# Autodesk Inventor assembly: 1977000 EAMM-A-D40-60P
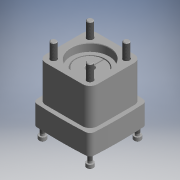
[picture p0: Inventor's stored thumbnail of the model, 180x180]
Saved by Autodesk Inventor 2017.3 (Build 213256000, 256)
## iProperties
Category: PARTsolutions
Company: FESTO
Part Number: 1977000 EAMM-A-D40-60P
Catalog Web Link: www.cadenas.de
Description: EAMM-A-axial kit
Vendor: FESTO
Document SubType Name: Assembly
Designer: partserver
Manufacturer: FESTO
Mass: 430 g
Surface Area: 514.373 cm^2
Volume: 141.907 cm^3
Density: 3.03016 g/cm^3
Title: 1977000 EAMM-A-D40-60P
Author: Cadenas PARTsolutions
Comments: axial kit
PSOL_IDENT_0: {ATYP=ASSISTANT},{DATA=script=$CADENAS_DATA/23d-libs/festo/webfesto.vbb&M_FAMILY=EAMM&M_GROUP=01&M_P
PSOL_IDENT_1: ARTNO=1977000&IDCODE1=EAMM-A-D40-60P&IDCODE2=&customer_number_cns=&MATES=1&LOD=HI&LOCKERP=0&SINGLEPA
PSOL_IDENT_2: RT=1}
NB: 1977000 EAMM-A-D40-60P
NN: EAMM-A
NT: axial kit
NBSYN: $TNR. $TYP.
LINA: 1977000 EAMM-A-D40-60P
CATALOG: Festo
TNR: 1977000
TYP: EAMM-A-D40-60P
CNSMASSEXACT: 0.43
SUPPLIER: FESTO
ARTICLENO: 1977000 EAMM-A-D40-60P
BOMINFO: 1977000 EAMM-A-D40-60P
CREATOR: CADENAS GmbH
## Documents named in this file (7)
- e:\temp\worker_10\temp\exporttempdir_3840_10_EllpH\format_0\1977000 EAMM-A-D40-60P.iam
- e:\temp\worker_10\temp\exporttempdir_3840_10_EllpH\format_0\552157 EAMK-A-D40-44A_C---(1O).ipt
- e:\temp\worker_10\temp\exporttempdir_3840_10_EllpH\format_0\DIN-912 - M6x30(F).ipt
- e:\temp\worker_10\temp\exporttempdir_3840_10_EllpH\format_0\1956846 EAMF-A-44C-60P(1A10).ipt
- e:\temp\worker_10\temp\exporttempdir_3840_10_EllpH\format_0\DIN-912 - M4x16(F).ipt
- e:\temp\worker_10\temp\exporttempdir_3840_10_EllpH\format_0\DIN-912 - M4x20(F).ipt
- e:\temp\worker_10\temp\exporttempdir_3840_10_EllpH\format_0\562682 EAMC-30-32-8-14.ipt
## Components (15 placed, 6 different names)
1. 552157 EAMK-A-D40-44A_C---(1O):1 — ZYL_SCHRAUBE_1_1_XY@1 <-> ANBAU_XY@2, ZYL_SCHRAUBE_1_1_Z@1 <-> ANBAU_Z@2, ZYL_SCHRAUBE_1_1_YZ@1 <-> ANBAU_YZ@2, ZYL_SCHRAUBE_1_2_XY@1 <-> ANBAU_XY@3, ZYL_SCHRAUBE_1_2_Z@1 <-> ANBAU_Z@3, ZYL_SCHRAUBE_1_2_YZ@1 <-> ANBAU_YZ@3, ZYL_SCHRAUBE_1_3_XY@1 <-> ANBAU_XY@4, ZYL_SCHRAUBE_1_3_Z@1 <-> ANBAU_Z@4, ZYL_SCHRAUBE_1_3_YZ@1 <-> ANBAU_YZ@4, ZYL_SCHRAUBE_1_4_XY@1 <-> ANBAU_XY@5, ZYL_SCHRAUBE_1_4_Z@1 <-> ANBAU_Z@5, ZYL_SCHRAUBE_1_4_YZ@1 <-> ANBAU_YZ@5
2. DIN-912 - M6x30(F):1 — ZYL_SCHRAUBE_1_1_XY@1 <-> ANBAU_XY@2, ZYL_SCHRAUBE_1_1_Z@1 <-> ANBAU_Z@2, ZYL_SCHRAUBE_1_1_YZ@1 <-> ANBAU_YZ@2
3. DIN-912 - M6x30(F):2 — ZYL_SCHRAUBE_1_2_XY@1 <-> ANBAU_XY@3, ZYL_SCHRAUBE_1_2_Z@1 <-> ANBAU_Z@3, ZYL_SCHRAUBE_1_2_YZ@1 <-> ANBAU_YZ@3
4. DIN-912 - M6x30(F):3 — ZYL_SCHRAUBE_1_3_XY@1 <-> ANBAU_XY@4, ZYL_SCHRAUBE_1_3_Z@1 <-> ANBAU_Z@4, ZYL_SCHRAUBE_1_3_YZ@1 <-> ANBAU_YZ@4
5. DIN-912 - M6x30(F):4 — ZYL_SCHRAUBE_1_4_XY@1 <-> ANBAU_XY@5, ZYL_SCHRAUBE_1_4_Z@1 <-> ANBAU_Z@5, ZYL_SCHRAUBE_1_4_YZ@1 <-> ANBAU_YZ@5
6. 1956846 EAMF-A-44C-60P(1A10):1 — ZYL_SCHRAUBE_1_1_XY@6 <-> ANBAU_XY@7, ZYL_SCHRAUBE_1_1_Z@6 <-> ANBAU_Z@7, ZYL_SCHRAUBE_1_1_YZ@6 <-> ANBAU_YZ@7, ZYL_SCHRAUBE_1_2_XY@6 <-> ANBAU_XY@8, ZYL_SCHRAUBE_1_2_Z@6 <-> ANBAU_Z@8, ZYL_SCHRAUBE_1_2_YZ@6 <-> ANBAU_YZ@8, ZYL_SCHRAUBE_1_3_XY@6 <-> ANBAU_XY@9, ZYL_SCHRAUBE_1_3_Z@6 <-> ANBAU_Z@9, ZYL_SCHRAUBE_1_3_YZ@6 <-> ANBAU_YZ@9, ZYL_SCHRAUBE_1_4_XY@6 <-> ANBAU_XY@10, ZYL_SCHRAUBE_1_4_Z@6 <-> ANBAU_Z@10, ZYL_SCHRAUBE_1_4_YZ@6 <-> ANBAU_YZ@10, ZYL_SCHRAUBE_2_1_XY@6 <-> ANBAU_XY@11, ZYL_SCHRAUBE_2_1_Z@6 <-> ANBAU_Z@11, ZYL_SCHRAUBE_2_1_YZ@6 <-> ANBAU_YZ@11, ZYL_SCHRAUBE_2_2_XY@6 <-> ANBAU_XY@12, ZYL_SCHRAUBE_2_2_Z@6 <-> ANBAU_Z@12, ZYL_SCHRAUBE_2_2_YZ@6 <-> ANBAU_YZ@12, ZYL_SCHRAUBE_2_3_XY@6 <-> ANBAU_XY@13, ZYL_SCHRAUBE_2_3_Z@6 <-> ANBAU_Z@13, ZYL_SCHRAUBE_2_3_YZ@6 <-> ANBAU_YZ@13, ZYL_SCHRAUBE_2_4_XY@6 <-> ANBAU_XY@14, ZYL_SCHRAUBE_2_4_Z@6 <-> ANBAU_Z@14, ZYL_SCHRAUBE_2_4_YZ@6 <-> ANBAU_YZ@14
7. DIN-912 - M4x16(F):1 — ZYL_SCHRAUBE_1_1_XY@6 <-> ANBAU_XY@7, ZYL_SCHRAUBE_1_1_Z@6 <-> ANBAU_Z@7, ZYL_SCHRAUBE_1_1_YZ@6 <-> ANBAU_YZ@7
8. DIN-912 - M4x16(F):2 — ZYL_SCHRAUBE_1_2_XY@6 <-> ANBAU_XY@8, ZYL_SCHRAUBE_1_2_Z@6 <-> ANBAU_Z@8, ZYL_SCHRAUBE_1_2_YZ@6 <-> ANBAU_YZ@8
9. DIN-912 - M4x16(F):3 — ZYL_SCHRAUBE_1_3_XY@6 <-> ANBAU_XY@9, ZYL_SCHRAUBE_1_3_Z@6 <-> ANBAU_Z@9, ZYL_SCHRAUBE_1_3_YZ@6 <-> ANBAU_YZ@9
10. DIN-912 - M4x16(F):4 — ZYL_SCHRAUBE_1_4_XY@6 <-> ANBAU_XY@10, ZYL_SCHRAUBE_1_4_Z@6 <-> ANBAU_Z@10, ZYL_SCHRAUBE_1_4_YZ@6 <-> ANBAU_YZ@10
11. DIN-912 - M4x20(F):1 — ZYL_SCHRAUBE_2_1_XY@6 <-> ANBAU_XY@11, ZYL_SCHRAUBE_2_1_Z@6 <-> ANBAU_Z@11, ZYL_SCHRAUBE_2_1_YZ@6 <-> ANBAU_YZ@11
12. DIN-912 - M4x20(F):2 — ZYL_SCHRAUBE_2_2_XY@6 <-> ANBAU_XY@12, ZYL_SCHRAUBE_2_2_Z@6 <-> ANBAU_Z@12, ZYL_SCHRAUBE_2_2_YZ@6 <-> ANBAU_YZ@12
13. DIN-912 - M4x20(F):3 — ZYL_SCHRAUBE_2_3_XY@6 <-> ANBAU_XY@13, ZYL_SCHRAUBE_2_3_Z@6 <-> ANBAU_Z@13, ZYL_SCHRAUBE_2_3_YZ@6 <-> ANBAU_YZ@13
14. DIN-912 - M4x20(F):4 — ZYL_SCHRAUBE_2_4_XY@6 <-> ANBAU_XY@14, ZYL_SCHRAUBE_2_4_Z@6 <-> ANBAU_Z@14, ZYL_SCHRAUBE_2_4_YZ@6 <-> ANBAU_YZ@14
15. 562682 EAMC-30-32-8-14:1
## Relationships (36: Mate 20, Angle 12, Flush 4)
- ZYL_SCHRAUBE_1_1_XY@1 <-> ANBAU_XY@2 [Flush]: 552157 EAMK-A-D40-44A_C---(1O):1 ↔ DIN-912 - M6x30(F):1
- ZYL_SCHRAUBE_1_1_Z@1 <-> ANBAU_Z@2 [Mate]: 552157 EAMK-A-D40-44A_C---(1O):1 ↔ DIN-912 - M6x30(F):1
- ZYL_SCHRAUBE_1_1_YZ@1 <-> ANBAU_YZ@2 [Angle] (0 deg): 552157 EAMK-A-D40-44A_C---(1O):1 ↔ DIN-912 - M6x30(F):1
- ZYL_SCHRAUBE_1_2_XY@1 <-> ANBAU_XY@3 [Flush]: 552157 EAMK-A-D40-44A_C---(1O):1 ↔ DIN-912 - M6x30(F):2
- ZYL_SCHRAUBE_1_2_Z@1 <-> ANBAU_Z@3 [Mate]: 552157 EAMK-A-D40-44A_C---(1O):1 ↔ DIN-912 - M6x30(F):2
- ZYL_SCHRAUBE_1_2_YZ@1 <-> ANBAU_YZ@3 [Angle] (0 deg): 552157 EAMK-A-D40-44A_C---(1O):1 ↔ DIN-912 - M6x30(F):2
- ZYL_SCHRAUBE_1_3_XY@1 <-> ANBAU_XY@4 [Flush]: 552157 EAMK-A-D40-44A_C---(1O):1 ↔ DIN-912 - M6x30(F):3
- ZYL_SCHRAUBE_1_3_Z@1 <-> ANBAU_Z@4 [Mate]: 552157 EAMK-A-D40-44A_C---(1O):1 ↔ DIN-912 - M6x30(F):3
- ZYL_SCHRAUBE_1_3_YZ@1 <-> ANBAU_YZ@4 [Angle] (0 deg): 552157 EAMK-A-D40-44A_C---(1O):1 ↔ DIN-912 - M6x30(F):3
- ZYL_SCHRAUBE_1_4_XY@1 <-> ANBAU_XY@5 [Flush]: 552157 EAMK-A-D40-44A_C---(1O):1 ↔ DIN-912 - M6x30(F):4
- ZYL_SCHRAUBE_1_4_Z@1 <-> ANBAU_Z@5 [Mate]: 552157 EAMK-A-D40-44A_C---(1O):1 ↔ DIN-912 - M6x30(F):4
- ZYL_SCHRAUBE_1_4_YZ@1 <-> ANBAU_YZ@5 [Angle] (0 deg): 552157 EAMK-A-D40-44A_C---(1O):1 ↔ DIN-912 - M6x30(F):4
- ZYL_SCHRAUBE_1_1_XY@6 <-> ANBAU_XY@7 [Mate]: 1956846 EAMF-A-44C-60P(1A10):1 ↔ DIN-912 - M4x16(F):1
- ZYL_SCHRAUBE_1_1_Z@6 <-> ANBAU_Z@7 [Mate]: 1956846 EAMF-A-44C-60P(1A10):1 ↔ DIN-912 - M4x16(F):1
- ZYL_SCHRAUBE_1_1_YZ@6 <-> ANBAU_YZ@7 [Angle] (0 deg): 1956846 EAMF-A-44C-60P(1A10):1 ↔ DIN-912 - M4x16(F):1
- ZYL_SCHRAUBE_1_2_XY@6 <-> ANBAU_XY@8 [Mate]: 1956846 EAMF-A-44C-60P(1A10):1 ↔ DIN-912 - M4x16(F):2
- ZYL_SCHRAUBE_1_2_Z@6 <-> ANBAU_Z@8 [Mate]: 1956846 EAMF-A-44C-60P(1A10):1 ↔ DIN-912 - M4x16(F):2
- ZYL_SCHRAUBE_1_2_YZ@6 <-> ANBAU_YZ@8 [Angle] (0 deg): 1956846 EAMF-A-44C-60P(1A10):1 ↔ DIN-912 - M4x16(F):2
- ZYL_SCHRAUBE_1_3_XY@6 <-> ANBAU_XY@9 [Mate]: 1956846 EAMF-A-44C-60P(1A10):1 ↔ DIN-912 - M4x16(F):3
- ZYL_SCHRAUBE_1_3_Z@6 <-> ANBAU_Z@9 [Mate]: 1956846 EAMF-A-44C-60P(1A10):1 ↔ DIN-912 - M4x16(F):3
- ZYL_SCHRAUBE_1_3_YZ@6 <-> ANBAU_YZ@9 [Angle] (0 deg): 1956846 EAMF-A-44C-60P(1A10):1 ↔ DIN-912 - M4x16(F):3
- ZYL_SCHRAUBE_1_4_XY@6 <-> ANBAU_XY@10 [Mate]: 1956846 EAMF-A-44C-60P(1A10):1 ↔ DIN-912 - M4x16(F):4
- ZYL_SCHRAUBE_1_4_Z@6 <-> ANBAU_Z@10 [Mate]: 1956846 EAMF-A-44C-60P(1A10):1 ↔ DIN-912 - M4x16(F):4
- ZYL_SCHRAUBE_1_4_YZ@6 <-> ANBAU_YZ@10 [Angle] (0 deg): 1956846 EAMF-A-44C-60P(1A10):1 ↔ DIN-912 - M4x16(F):4
- ZYL_SCHRAUBE_2_1_XY@6 <-> ANBAU_XY@11 [Mate]: 1956846 EAMF-A-44C-60P(1A10):1 ↔ DIN-912 - M4x20(F):1
- ZYL_SCHRAUBE_2_1_Z@6 <-> ANBAU_Z@11 [Mate]: 1956846 EAMF-A-44C-60P(1A10):1 ↔ DIN-912 - M4x20(F):1
- ZYL_SCHRAUBE_2_1_YZ@6 <-> ANBAU_YZ@11 [Angle] (0 deg): 1956846 EAMF-A-44C-60P(1A10):1 ↔ DIN-912 - M4x20(F):1
- ZYL_SCHRAUBE_2_2_XY@6 <-> ANBAU_XY@12 [Mate]: 1956846 EAMF-A-44C-60P(1A10):1 ↔ DIN-912 - M4x20(F):2
- ZYL_SCHRAUBE_2_2_Z@6 <-> ANBAU_Z@12 [Mate]: 1956846 EAMF-A-44C-60P(1A10):1 ↔ DIN-912 - M4x20(F):2
- ZYL_SCHRAUBE_2_2_YZ@6 <-> ANBAU_YZ@12 [Angle] (0 deg): 1956846 EAMF-A-44C-60P(1A10):1 ↔ DIN-912 - M4x20(F):2
- ZYL_SCHRAUBE_2_3_XY@6 <-> ANBAU_XY@13 [Mate]: 1956846 EAMF-A-44C-60P(1A10):1 ↔ DIN-912 - M4x20(F):3
- ZYL_SCHRAUBE_2_3_Z@6 <-> ANBAU_Z@13 [Mate]: 1956846 EAMF-A-44C-60P(1A10):1 ↔ DIN-912 - M4x20(F):3
- ZYL_SCHRAUBE_2_3_YZ@6 <-> ANBAU_YZ@13 [Angle] (0 deg): 1956846 EAMF-A-44C-60P(1A10):1 ↔ DIN-912 - M4x20(F):3
- ZYL_SCHRAUBE_2_4_XY@6 <-> ANBAU_XY@14 [Mate]: 1956846 EAMF-A-44C-60P(1A10):1 ↔ DIN-912 - M4x20(F):4
- ZYL_SCHRAUBE_2_4_Z@6 <-> ANBAU_Z@14 [Mate]: 1956846 EAMF-A-44C-60P(1A10):1 ↔ DIN-912 - M4x20(F):4
- ZYL_SCHRAUBE_2_4_YZ@6 <-> ANBAU_YZ@14 [Angle] (0 deg): 1956846 EAMF-A-44C-60P(1A10):1 ↔ DIN-912 - M4x20(F):4
